# Autodesk Inventor assembly: !Hook
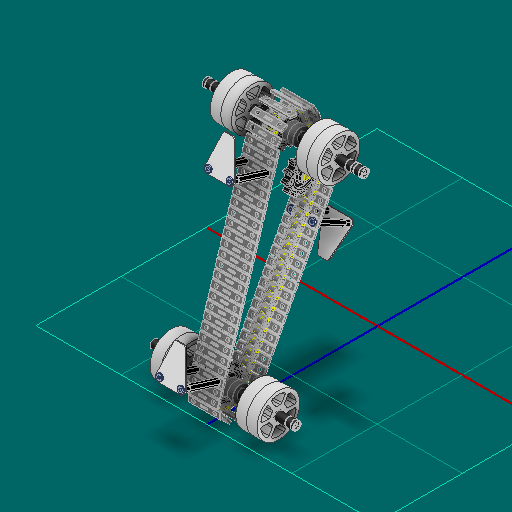
[picture p0: Inventor's stored thumbnail of the model, 512x512]
Saved by Autodesk Inventor 2025 (Build 290162000, 162)
## iProperties
Created: 2024-10-20
Part Number: !Hook
Document SubType Name: Assembly
Designer: Averey Ku
Author: Averey Ku
## Documents named in this file (14)
- C:\Users\avere\VEX\High Stakes\CAD\V2\Hook\!Hook.iam
- C:\Users\avere\VEX\High Stakes\CAD\V2\Hook\Chain.iam
- C:\Users\avere\VEX\High Stakes\CAD\V2\Hook\Custom Parts\Hook Gusset.ipt
- C:\Users\avere\VEX\High Stakes\CAD\ROBOPROS-CAD-Inventor\Structure\Standoff\Standoff .25.ipt
- C:\Users\avere\VEX\High Stakes\CAD\ROBOPROS-CAD-Inventor\Structure\Standoff\Standoff 1.50.ipt
- C:\Users\avere\VEX\High Stakes\CAD\ROBOPROS-CAD-Inventor\Structure\Hardware\Screw Shoulder Robosource\SScrew Shoulder Smooth .500 x .04.ipt
- C:\Users\avere\VEX\High Stakes\CAD\ROBOPROS-CAD-Inventor\Motion\Sprockets\9P Sprocket\9P 12T Sprocket, No Insert.iam
- C:\Users\avere\VEX\High Stakes\CAD\V2\Hook\Roller Shaft.iam
- C:\Users\avere\VEX\High Stakes\CAD\ROBOPROS-CAD-Inventor\Structure\Standoff.ipt
- C:\Users\avere\VEX\High Stakes\CAD\ROBOPROS-CAD-Inventor\Structure\Hardware\Screw Shoulder Robosource.ipt
- C:\Users\avere\VEX\High Stakes\CAD\ROBOPROS-CAD-Inventor\Motion\Sprockets\9P Sprocket.iam
- C:\Users\avere\VEX\High Stakes\CAD\ROBOPROS-CAD-Inventor\Motion\Shaft HS\HS Spacer\HSpacer .1250.ipt
- C:\Users\avere\VEX\High Stakes\CAD\ROBOPROS-CAD-Inventor\Motion\Shaft HS\HS Spacer.ipt
- C:\Users\avere\VEX\High Stakes\CAD\ROBOPROS-CAD-Inventor\Motion\Shaft HS\HS Spacer\HSpacer .2500.ipt
## Components (35 placed, 9 different names)
1. Chain:1 [sub-assembly] — Insert:1, Insert:4, Insert:9, Insert:10, Insert:20, Mate:5, Insert:31, Mate:6, Mate:7, Mate:8, Mate:9
2. Roller Shaft:1 [sub-assembly] — Flush:1, Mate:7, Mate:10
3. Roller Shaft:2 [sub-assembly] — Flush:2, Mate:8, Insert:33, Insert:35
4. 9P 12T Sprocket, No Insert:1 [sub-assembly] — Mate:9, Mate:10
5. HSpacer .1250:1 — Insert:32
6. HSpacer .2500:2 — Insert:32, Insert:33
7. HSpacer .1250:3
8. HSpacer .2500:4 — Insert:35
9. Hook Gusset:1 — Insert:3, Insert:6, Insert:7, Insert:8
10. Standoff .25:1 — Insert:5, Insert:6
11. Standoff 1.50:2 — Insert:4, Insert:5
12. Standoff .25:3 — Insert:2, Insert:3
13. Standoff 1.50:4 — Insert:1, Insert:2
14. SScrew Shoulder Smooth .500 x .04:1 — Insert:8
15. SScrew Shoulder Smooth .500 x .04:2 — Insert:7
16. SScrew Shoulder Smooth .500 x .04:3 — Insert:10
17. SScrew Shoulder Smooth .500 x .04:4 — Insert:9
18. Hook Gusset:2
19. Standoff .25:5
20. Standoff 1.50:6 — Insert:20, Insert:21
21. Standoff .25:7
22. Standoff 1.50:8 — Mate:5, Insert:22
23. SScrew Shoulder Smooth .500 x .04:5
24. SScrew Shoulder Smooth .500 x .04:6
25. SScrew Shoulder Smooth .500 x .04:8 — Insert:22
26. SScrew Shoulder Smooth .500 x .04:7 — Insert:21
27. Hook Gusset:3
28. Standoff .25:9
29. Standoff 1.50:10 — Mate:6
30. Standoff .25:11
31. Standoff 1.50:12 — Insert:31
32. SScrew Shoulder Smooth .500 x .04:9
33. SScrew Shoulder Smooth .500 x .04:10
34. SScrew Shoulder Smooth .500 x .04:11
35. SScrew Shoulder Smooth .500 x .04:12
## Relationships (40: Insert 32, Mate 6, Flush 2)
- Insert:1: Chain:1 ↔ Standoff 1.50:4
- Insert:2: Standoff .25:3 ↔ Standoff 1.50:4
- Insert:3: Hook Gusset:1 ↔ Standoff .25:3
- Insert:4: Chain:1 ↔ Standoff 1.50:2
- Insert:5: Standoff .25:1 ↔ Standoff 1.50:2
- Insert:6: Hook Gusset:1 ↔ Standoff .25:1
- Insert:7: Hook Gusset:1 ↔ SScrew Shoulder Smooth .500 x .04:2
- Insert:8: Hook Gusset:1 ↔ SScrew Shoulder Smooth .500 x .04:1
- Insert:9: Chain:1 ↔ SScrew Shoulder Smooth .500 x .04:4
- Insert:10: Chain:1 ↔ SScrew Shoulder Smooth .500 x .04:3
- [Insert]: Standoff .25:7 ↔ Standoff 1.50:8
- [Insert]: Hook Gusset:2 ↔ Standoff .25:7
- [Insert]: Standoff .25:5 ↔ Standoff 1.50:6
- [Insert]: Hook Gusset:2 ↔ Standoff .25:5
- [Insert]: Hook Gusset:2 ↔ SScrew Shoulder Smooth .500 x .04:6
- [Insert]: Hook Gusset:2 ↔ SScrew Shoulder Smooth .500 x .04:5
- Insert:20: Chain:1 ↔ Standoff 1.50:6
- Mate:5: Chain:1 ↔ Standoff 1.50:8
- Insert:21 (3.175 mm): Standoff 1.50:6 ↔ SScrew Shoulder Smooth .500 x .04:7
- Insert:22 (3.175 mm): Standoff 1.50:8 ↔ SScrew Shoulder Smooth .500 x .04:8
- [Insert]: Standoff .25:11 ↔ Standoff 1.50:12
- [Insert]: Hook Gusset:3 ↔ Standoff .25:11
- [Insert]: Standoff .25:9 ↔ Standoff 1.50:10
- [Insert]: Hook Gusset:3 ↔ Standoff .25:9
- [Insert]: Hook Gusset:3 ↔ SScrew Shoulder Smooth .500 x .04:10
- [Insert]: Hook Gusset:3 ↔ SScrew Shoulder Smooth .500 x .04:9
- [Insert] (3.175 mm): Standoff 1.50:10 ↔ SScrew Shoulder Smooth .500 x .04:11
- [Insert] (3.175 mm): Standoff 1.50:12 ↔ SScrew Shoulder Smooth .500 x .04:12
- Insert:31: Chain:1 ↔ Standoff 1.50:12
- Mate:6: Chain:1 ↔ Standoff 1.50:10
- Flush:1 (6.35 mm): Roller Shaft:1
- Mate:7: Chain:1 ↔ Roller Shaft:1
- Flush:2 (6.35 mm): Roller Shaft:2
- Mate:8: Chain:1 ↔ Roller Shaft:2
- Mate:9: Chain:1 ↔ 9P 12T Sprocket, No Insert:1
- Mate:10: Roller Shaft:1 ↔ 9P 12T Sprocket, No Insert:1
- Insert:32: HSpacer .1250:1 ↔ HSpacer .2500:2
- Insert:33: Roller Shaft:2 ↔ HSpacer .2500:2
- [Insert]: HSpacer .1250:3 ↔ HSpacer .2500:4
- Insert:35: Roller Shaft:2 ↔ HSpacer .2500:4
## Named parameters: d16_d1 = 0 mm, d17_d2 = 0 mm, d18_d4 = 0 mm, d19_d5 = 0 mm, d20_d6 = 0 mm, d21_d7 = 0 mm, d30_d28 = 3.175 mm, d31_d29 = 3.175 mm, d32_d16_d1 = 0 mm, d33_d17_d2 = 0 mm, d34_d18_d4 = 0 mm, d35_d19_d5 = 0 mm, d36_d20_d6 = 0 mm, d37_d21_d7 = 0 mm, d73_d71 = 0 mm
